# Autodesk Inventor assembly: Bench
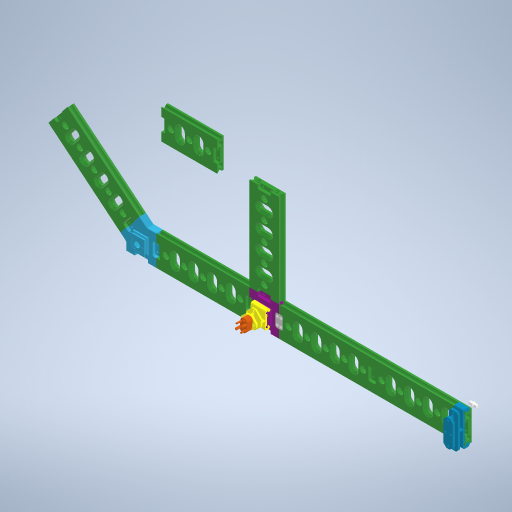
[picture p0: Inventor's stored thumbnail of the model, 512x512]
Saved by Autodesk Inventor 2023.1 (Build 271208000, 208)
## iProperties
Created: 2023-06-05
Part Number: Bench
Document SubType Name: Assembly
Designer: hello
Author: hello
## Documents named in this file (10)
- D:\Git\PrintableOpticsBench\Bench.iam
- D:\Git\PrintableOpticsBench\Rail-250MM.ipt
- D:\Git\PrintableOpticsBench\Rail-Square.ipt
- D:\Git\PrintableOpticsBench\MicroRail-FlextureBase.ipt
- D:\Git\PrintableOpticsBench\RailPlug.ipt
- D:\Git\PrintableOpticsBench\RailTab.ipt
- D:\Git\PrintableOpticsBench\MicroRail-FlextureBase-CubeAttachment.ipt
- D:\Git\PrintableOpticsBench\Rail-FlextureBase.ipt
- D:\Git\PrintableOpticsBench\Rail-Angle140.66.ipt
- D:\Git\PrintableOpticsBench\Rail-150MM.ipt
## Components (13 placed, 9 different names)
1. Rail-250MM:1 — Mate:10, Mate:11, Mate:12
2. Rail-250MM:2 — Mate:7, Mate:8, Mate:9, Mate:18, Flush:2, Flush:3
3. Rail-250MM:3 — Mate:4, Mate:5, Mate:6, Mate:7, Mate:8, Mate:9
4. Rail-250MM:4 — Mate:1, Mate:2, Mate:3, Mate:23, Mate:24, Mate:25
5. Rail-Square:1 — Mate:1, Mate:2, Mate:3, Mate:4, Mate:5, Mate:6, Mate:10, Mate:11, Mate:12, Mate:15, Mate:16, Mate:17, Mate:19, Mate:20
6. MicroRail-FlextureBase:1 — Flush:1, Mate:19, Mate:20, Mate:21, Mate:22
7. RailPlug:1
8. RailTab:1 — Mate:15, Mate:16, Mate:17
9. MicroRail-FlextureBase-CubeAttachment:1 — Flush:1, Mate:21, Mate:22
10. Rail-FlextureBase:1 — Mate:18, Flush:2, Flush:3
11. Rail-Angle140.66:1 — Mate:23, Mate:24, Mate:25, Mate:26, Mate:27, Mate:28
12. Rail-250MM:5 — Mate:26, Mate:27, Mate:28
13. Rail-150MM:1
## Relationships (29: Mate 26, Flush 3)
- Mate:1: Rail-250MM:4 ↔ Rail-Square:1
- Mate:2: Rail-250MM:4 ↔ Rail-Square:1
- Mate:3: Rail-250MM:4 ↔ Rail-Square:1
- Mate:4: Rail-250MM:3 ↔ Rail-Square:1
- Mate:5: Rail-250MM:3 ↔ Rail-Square:1
- Mate:6: Rail-250MM:3 ↔ Rail-Square:1
- Mate:7: Rail-250MM:2 ↔ Rail-250MM:3
- Mate:8: Rail-250MM:2 ↔ Rail-250MM:3
- Mate:9: Rail-250MM:2 ↔ Rail-250MM:3
- Mate:10: Rail-250MM:1 ↔ Rail-Square:1
- Mate:11: Rail-250MM:1 ↔ Rail-Square:1
- Mate:12: Rail-250MM:1 ↔ Rail-Square:1
- Mate:15: Rail-Square:1 ↔ RailTab:1
- Mate:16: Rail-Square:1 ↔ RailTab:1
- Mate:17: Rail-Square:1 ↔ RailTab:1
- Flush:1: MicroRail-FlextureBase:1 ↔ MicroRail-FlextureBase-CubeAttachment:1
- Mate:18: Rail-250MM:2 ↔ Rail-FlextureBase:1
- Flush:2: Rail-250MM:2 ↔ Rail-FlextureBase:1
- Flush:3: Rail-250MM:2 ↔ Rail-FlextureBase:1
- Mate:19: Rail-Square:1 ↔ MicroRail-FlextureBase:1
- Mate:20: Rail-Square:1 ↔ MicroRail-FlextureBase:1
- Mate:21: MicroRail-FlextureBase:1 ↔ MicroRail-FlextureBase-CubeAttachment:1
- Mate:22: MicroRail-FlextureBase:1 ↔ MicroRail-FlextureBase-CubeAttachment:1
- Mate:23: Rail-250MM:4 ↔ Rail-Angle140.66:1
- Mate:24: Rail-250MM:4 ↔ Rail-Angle140.66:1
- Mate:25: Rail-250MM:4 ↔ Rail-Angle140.66:1
- Mate:26: Rail-Angle140.66:1 ↔ Rail-250MM:5
- Mate:27: Rail-Angle140.66:1 ↔ Rail-250MM:5
- Mate:28: Rail-Angle140.66:1 ↔ Rail-250MM:5
